# Autodesk Inventor assembly: test-model-1
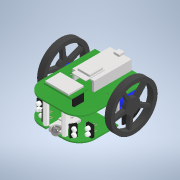
[picture p0: Inventor's stored thumbnail of the model, 180x180]
Saved by Autodesk Inventor 2022 (Build 260153000, 153)
## iProperties
Created: 2024-05-30
Part Number: test-model-1
Document SubType Name: Assembly
Designer: yamashita1
Author: yamashita1
## Documents named in this file (13)
- G:\マイドライブ\project\micro-mouse\3D-Model\test-model-1.iam
- G:\マイドライブ\project\micro-mouse\3D-Model\PCB-Bottom.ipt
- G:\マイドライブ\project\micro-mouse\3D-Model\FS90R.ipt
- G:\マイドライブ\project\micro-mouse\3D-Model\FS90R-W.ipt
- G:\マイドライブ\project\micro-mouse\3D-Model\PCB-main.ipt
- G:\マイドライブ\project\micro-mouse\3D-Model\FS90-Mount2.ipt
- G:\マイドライブ\project\micro-mouse\3D-Model\FS90-Mount2-Mirror.ipt
- G:\マイドライブ\project\micro-mouse\3D-Model\Photo-Sensor.iam
- G:\マイドライブ\project\micro-mouse\3D-Model\ESP32-DevKitC.ipt
- G:\マイドライブ\project\micro-mouse\3D-Model\TAMIYA-70246.ipt
- G:\マイドライブ\project\micro-mouse\3D-Model\PCB-EncoderSensor.ipt
- G:\マイドライブ\project\micro-mouse\3D-Model\Spacer-M3H28.ipt
- G:\マイドライブ\project\micro-mouse\3D-Model\PCB-AE-AQM0802.ipt
## Components (21 placed, 12 different names)
1. PCB-Bottom:1 — メイト:8, メイト:10, フラッシュ:6, メイト:13, メイト:14, メイト:16, フラッシュ:10, メイト:41, メイト:50, メイト:51, メイト:52, メイト:53, メイト:54
2. FS90R:1 — 回転:1, メイト:8, フラッシュ:8, メイト:15
3. FS90R:2 — 回転:2, メイト:10, フラッシュ:9, メイト:17
4. FS90R-W:1 — 回転:1
5. FS90R-W:2 — 回転:2
6. PCB-main:1 — フラッシュ:6, メイト:13, メイト:27, メイト:28, メイト:29, メイト:30, メイト:33, メイト:34, フラッシュ:10, メイト:42, メイト:43, メイト:44, メイト:45, メイト:46, メイト:47, メイト:48, メイト:49
7. FS90-Mount2:1 — フラッシュ:8, メイト:14, メイト:15, メイト:35, メイト:36, メイト:37, メイト:50, メイト:51
8. FS90-Mount2-Mirror:1 — フラッシュ:9, メイト:16, メイト:17, メイト:38, メイト:39, メイト:40, メイト:52, メイト:53
9. Photo-Sensor:1 [sub-assembly] — メイト:27
10. Photo-Sensor:2 [sub-assembly] — メイト:28
11. Photo-Sensor:3 [sub-assembly] — メイト:29
12. Photo-Sensor:4 [sub-assembly] — メイト:30
13. ESP32-DevKitC:1 — メイト:41
14. TAMIYA-70246:1 — メイト:33, メイト:34
15. PCB-EncoderSensor:1 — メイト:35, メイト:36, メイト:37
16. PCB-EncoderSensor:2 — メイト:38, メイト:39, メイト:40
17. Spacer-M3H28:1 — メイト:42, メイト:47
18. Spacer-M3H28:2 — メイト:43, メイト:46
19. Spacer-M3H28:3 — メイト:45, メイト:48
20. Spacer-M3H28:4 — メイト:44, メイト:49
21. PCB-AE-AQM0802:1 — メイト:54
## Relationships (39: Mate 33, Flush 4, RevoluteJoint 2)
- 回転:1 [RevoluteJoint]: FS90R:1 ↔ FS90R-W:1
- 回転:2 [RevoluteJoint]: FS90R:2 ↔ FS90R-W:2
- メイト:8 [Mate]: PCB-Bottom:1 ↔ FS90R:1
- メイト:10 [Mate]: PCB-Bottom:1 ↔ FS90R:2
- フラッシュ:6 [Flush]: PCB-Bottom:1 ↔ PCB-main:1
- メイト:13 [Mate] (28 mm): PCB-Bottom:1 ↔ PCB-main:1
- フラッシュ:8 [Flush]: FS90R:1 ↔ FS90-Mount2:1
- メイト:14 [Mate]: PCB-Bottom:1 ↔ FS90-Mount2:1
- メイト:15 [Mate] (0.2 mm): FS90R:1 ↔ FS90-Mount2:1
- フラッシュ:9 [Flush]: FS90R:2 ↔ FS90-Mount2-Mirror:1
- メイト:16 [Mate]: PCB-Bottom:1 ↔ FS90-Mount2-Mirror:1
- メイト:17 [Mate] (0.2 mm): FS90R:2 ↔ FS90-Mount2-Mirror:1
- メイト:27 [Mate]: PCB-main:1 ↔ Photo-Sensor:1
- メイト:28 [Mate]: PCB-main:1 ↔ Photo-Sensor:2
- メイト:29 [Mate]: PCB-main:1 ↔ Photo-Sensor:3
- メイト:30 [Mate]: PCB-main:1 ↔ Photo-Sensor:4
- メイト:33 [Mate]: PCB-main:1 ↔ TAMIYA-70246:1
- メイト:34 [Mate]: PCB-main:1 ↔ TAMIYA-70246:1
- メイト:35 [Mate]: FS90-Mount2:1 ↔ PCB-EncoderSensor:1
- メイト:36 [Mate]: FS90-Mount2:1 ↔ PCB-EncoderSensor:1
- メイト:37 [Mate]: FS90-Mount2:1 ↔ PCB-EncoderSensor:1
- メイト:38 [Mate]: FS90-Mount2-Mirror:1 ↔ PCB-EncoderSensor:2
- メイト:39 [Mate]: FS90-Mount2-Mirror:1 ↔ PCB-EncoderSensor:2
- メイト:40 [Mate]: FS90-Mount2-Mirror:1 ↔ PCB-EncoderSensor:2
- フラッシュ:10 [Flush]: PCB-Bottom:1 ↔ PCB-main:1
- メイト:41 [Mate]: PCB-Bottom:1 ↔ ESP32-DevKitC:1
- メイト:42 [Mate]: PCB-main:1 ↔ Spacer-M3H28:1
- メイト:43 [Mate]: PCB-main:1 ↔ Spacer-M3H28:2
- メイト:44 [Mate]: PCB-main:1 ↔ Spacer-M3H28:4
- メイト:45 [Mate]: PCB-main:1 ↔ Spacer-M3H28:3
- メイト:46 [Mate]: PCB-main:1 ↔ Spacer-M3H28:2
- メイト:47 [Mate]: PCB-main:1 ↔ Spacer-M3H28:1
- メイト:48 [Mate]: PCB-main:1 ↔ Spacer-M3H28:3
- メイト:49 [Mate]: PCB-main:1 ↔ Spacer-M3H28:4
- メイト:50 [Mate]: PCB-Bottom:1 ↔ FS90-Mount2:1
- メイト:51 [Mate]: PCB-Bottom:1 ↔ FS90-Mount2:1
- メイト:52 [Mate]: PCB-Bottom:1 ↔ FS90-Mount2-Mirror:1
- メイト:53 [Mate]: PCB-Bottom:1 ↔ FS90-Mount2-Mirror:1
- メイト:54 [Mate]: PCB-Bottom:1 ↔ PCB-AE-AQM0802:1
